# Autodesk Inventor assembly: Assembly1
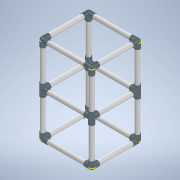
[picture p0: Inventor's stored thumbnail of the model, 180x180]
Saved by Autodesk Inventor 2020 (Build 240168000, 168)
## iProperties
Created: 2020-01-17
Part Number: Assembly1
Document SubType Name: Assembly
Designer: Gebruiker
Author: Gebruiker
## Documents named in this file (5)
- \\Festina.edu.adm.local\jonas.vandenborne$\Downloads\Assembly1.iam
- \\Festina.edu.adm.local\jonas.vandenborne$\Downloads\hoek drieweg.ipt
- \\Festina.edu.adm.local\jonas.vandenborne$\Downloads\buis lang.ipt
- \\Festina.edu.adm.local\jonas.vandenborne$\Downloads\buis.ipt
- \\Festina.edu.adm.local\jonas.vandenborne$\Downloads\hoek vierweg.ipt
## Components (28 placed, 4 different names)
1. buis lang:1 — Cylindrical:1, Rotational:1, Cylindrical:16, Cylindrical:30
2. hoek drieweg:1 — Mate:1, Mate:2, Cylindrical:1, Rotational:1, Cylindrical:2, Rotational:2, Cylindrical:3, Rotational:3
3. buis:1 — Cylindrical:3, Rotational:3, Cylindrical:4, Rotational:4
4. buis:2 — Cylindrical:6, Rotational:6, Cylindrical:7, Rotational:7
5. buis:3 — Cylindrical:5, Rotational:5, Cylindrical:8
6. buis:4 — Cylindrical:2, Rotational:2, Rigid:1
7. hoek drieweg:2 — Cylindrical:7, Rotational:7, Cylindrical:8, Cylindrical:12, Rotational:8
8. hoek drieweg:3 — Rigid:1, Cylindrical:6, Rotational:6, Cylindrical:20, Rotational:14
9. hoek drieweg:4 — Cylindrical:4, Rotational:4, Cylindrical:5, Rotational:5, Cylindrical:10, Rotational:9, Mate:3
10. buis lang:3 — Cylindrical:10, Rotational:9, Cylindrical:15, Rotational:12, Cylindrical:29
11. buis lang:4 — Cylindrical:12, Rotational:8, Cylindrical:18, Rotational:13, Cylindrical:28
12. hoek drieweg:6 — Cylindrical:15, Cylindrical:17, Rotational:11, Rotational:12, Cylindrical:24
13. hoek drieweg:7 — Cylindrical:16, Cylindrical:22, Rotational:16, Cylindrical:23, Rotational:17
14. hoek drieweg:8 — Cylindrical:18, Rotational:13, Cylindrical:19, Cylindrical:26
15. buis:5 — Cylindrical:17, Rotational:11, Cylindrical:19
16. buis:6 — Cylindrical:23, Rotational:17
17. buis:7 — Cylindrical:25, Cylindrical:26, Rotational:18
18. buis:8 — Cylindrical:22, Rotational:16, Cylindrical:24
19. hoek drieweg:9 — Cylindrical:21, Rotational:15, Cylindrical:25, Rotational:18
20. buis lang:5 — Cylindrical:20, Rotational:14, Cylindrical:21, Rotational:15, Cylindrical:27
21. hoek vierweg:1 — Cylindrical:27, Rotational:19, Rotational:22
22. buis:9 — Rotational:25
23. buis:10 — Rotational:22, Rotational:23
24. buis:11 — Rotational:19, Rotational:20
25. buis:12 — Rotational:21, Rotational:24
26. hoek vierweg:2 — Cylindrical:28, Rotational:20, Rotational:21
27. hoek vierweg:4 — Cylindrical:29, Rotational:24, Mate:3
28. hoek vierweg:5 — Cylindrical:30, Rotational:23, Rotational:25
## Relationships (54: CylindricalJoint 26, RevoluteJoint 24, Mate 3, WeldJoint 1)
- Mate:1: hoek drieweg:1
- Mate:2: hoek drieweg:1
- Cylindrical:1: buis lang:1 ↔ hoek drieweg:1
- Rotational:1 [RevoluteJoint]: buis lang:1 ↔ hoek drieweg:1
- Cylindrical:2: hoek drieweg:1 ↔ buis:4
- Rotational:2 [RevoluteJoint]: hoek drieweg:1 ↔ buis:4
- Cylindrical:3: hoek drieweg:1 ↔ buis:1
- Rotational:3 [RevoluteJoint]: hoek drieweg:1 ↔ buis:1
- Cylindrical:4: buis:1 ↔ hoek drieweg:4
- Rigid:1 [WeldJoint]: buis:4 ↔ hoek drieweg:3
- Rotational:4 [RevoluteJoint]: buis:1 ↔ hoek drieweg:4
- Cylindrical:5: buis:3 ↔ hoek drieweg:4
- Rotational:5 [RevoluteJoint]: buis:3 ↔ hoek drieweg:4
- Cylindrical:6: buis:2 ↔ hoek drieweg:3
- Rotational:6 [RevoluteJoint]: buis:2 ↔ hoek drieweg:3
- Cylindrical:7: buis:2 ↔ hoek drieweg:2
- Rotational:7 [RevoluteJoint]: buis:2 ↔ hoek drieweg:2
- Cylindrical:8: buis:3 ↔ hoek drieweg:2
- Cylindrical:10: hoek drieweg:4 ↔ buis lang:3
- Cylindrical:12: hoek drieweg:2 ↔ buis lang:4
- Rotational:8 [RevoluteJoint]: hoek drieweg:2 ↔ buis lang:4
- Rotational:9 [RevoluteJoint]: hoek drieweg:4 ↔ buis lang:3
- Cylindrical:15: buis lang:3 ↔ hoek drieweg:6
- Cylindrical:16: buis lang:1 ↔ hoek drieweg:7
- Cylindrical:17: hoek drieweg:6 ↔ buis:5
- Rotational:11 [RevoluteJoint]: hoek drieweg:6 ↔ buis:5
- Rotational:12 [RevoluteJoint]: buis lang:3 ↔ hoek drieweg:6
- Cylindrical:18: buis lang:4 ↔ hoek drieweg:8
- Rotational:13 [RevoluteJoint]: buis lang:4 ↔ hoek drieweg:8
- Cylindrical:19: hoek drieweg:8 ↔ buis:5
- Cylindrical:20: hoek drieweg:3 ↔ buis lang:5
- Rotational:14 [RevoluteJoint]: hoek drieweg:3 ↔ buis lang:5
- Cylindrical:21: hoek drieweg:9 ↔ buis lang:5
- Rotational:15 [RevoluteJoint]: hoek drieweg:9 ↔ buis lang:5
- Cylindrical:22: hoek drieweg:7 ↔ buis:8
- Rotational:16 [RevoluteJoint]: hoek drieweg:7 ↔ buis:8
- Cylindrical:23: hoek drieweg:7 ↔ buis:6
- Rotational:17 [RevoluteJoint]: hoek drieweg:7 ↔ buis:6
- Cylindrical:24: hoek drieweg:6 ↔ buis:8
- Cylindrical:25: buis:7 ↔ hoek drieweg:9
- Cylindrical:26: hoek drieweg:8 ↔ buis:7
- Rotational:18 [RevoluteJoint]: buis:7 ↔ hoek drieweg:9
- Cylindrical:27: buis lang:5 ↔ hoek vierweg:1
- Rotational:19 [RevoluteJoint]: hoek vierweg:1 ↔ buis:11
- Cylindrical:28: buis lang:4 ↔ hoek vierweg:2
- Rotational:20 [RevoluteJoint]: buis:11 ↔ hoek vierweg:2
- Rotational:21 [RevoluteJoint]: buis:12 ↔ hoek vierweg:2
- Cylindrical:29: buis lang:3 ↔ hoek vierweg:4
- Rotational:22 [RevoluteJoint]: hoek vierweg:1 ↔ buis:10
- Cylindrical:30: buis lang:1 ↔ hoek vierweg:5
- Rotational:23 [RevoluteJoint]: buis:10 ↔ hoek vierweg:5
- Rotational:24 [RevoluteJoint]: buis:12 ↔ hoek vierweg:4
- Rotational:25 [RevoluteJoint]: buis:9 ↔ hoek vierweg:5
- Mate:3 (155 mm): hoek drieweg:4 ↔ hoek vierweg:4
